# Autodesk Inventor assembly: 100-10-FRAME-TOP
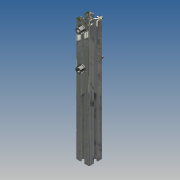
[picture p0: Inventor's stored thumbnail of the model, 180x180]
Saved by Autodesk Inventor 2018.2 (Build 222227000, 227)
## iProperties
Manager: feesmrt
Company: FRANCOR
Part Number: 100-10-FRAME-TOP
Project: Rescue Robot
Cost Center: -
Material: Generisch
Document SubType Name: Assembly
Designer: feesmrt
Engineer: feesmrt
Authority: feesmrt
Subject: Rescue Robot
Author: feesmrt
Revision Number: 1
## Documents named in this file (4)
- C:\Users\feesmrt\Documents\FRANC0R\CAD\02-Rocker-Bogie-Robot\100-CHASSIS\10-FRAME\100-10-FRAME-TOP.iam
- C:\Users\feesmrt\Documents\FRANC0R\CAD\02-Rocker-Bogie-Robot\100-CHASSIS\10-FRAME\100-10-FRAME-PROFILE-TOP-L-01.ipt
- C:\Users\feesmrt\Documents\FRANC0R\CAD\02-Rocker-Bogie-Robot\100-CHASSIS\10-FRAME\100-10-FRAME-ROCKER-SCREW-01.iam
- C:\Users\feesmrt\Documents\FRANC0R\CAD\02-Rocker-Bogie-Robot\900-COMPONENTS\900-40-SCREWS\900-40-SCREWS-ISO7380_M8x16.ipt
## Components (4 placed, 3 different names)
1. 100-10-FRAME-PROFILE-TOP-L-01:1 — Passend:1, Passend:2, Passend:3, Passend:4, Passend:5, Passend:6
2. 100-10-FRAME-ROCKER-SCREW-01:1 [sub-assembly] — Passend:1, Passend:3
3. 100-10-FRAME-ROCKER-SCREW-01:2 [sub-assembly] — Passend:2, Passend:4
4. 900-40-SCREWS-ISO7380_M8x16:1 — Passend:5, Passend:6
## Relationships (6: Mate 6)
- Passend:1 [Mate]: 100-10-FRAME-PROFILE-TOP-L-01:1 ↔ 100-10-FRAME-ROCKER-SCREW-01:1
- Passend:2 [Mate]: 100-10-FRAME-PROFILE-TOP-L-01:1 ↔ 100-10-FRAME-ROCKER-SCREW-01:2
- Passend:3 [Mate]: 100-10-FRAME-PROFILE-TOP-L-01:1 ↔ 100-10-FRAME-ROCKER-SCREW-01:1
- Passend:4 [Mate]: 100-10-FRAME-PROFILE-TOP-L-01:1 ↔ 100-10-FRAME-ROCKER-SCREW-01:2
- Passend:5 [Mate]: 100-10-FRAME-PROFILE-TOP-L-01:1 ↔ 900-40-SCREWS-ISO7380_M8x16:1
- Passend:6 [Mate] (2.8 mm): 100-10-FRAME-PROFILE-TOP-L-01:1 ↔ 900-40-SCREWS-ISO7380_M8x16:1
